# Autodesk Inventor assembly: Assembly1
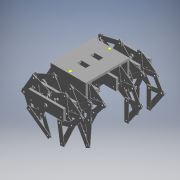
[picture p0: Inventor's stored thumbnail of the model, 180x180]
Saved by Autodesk Inventor 2018 (Build 220112000, 112)
## iProperties
Created: 2018-10-06
Part Number: Assembly1
Document SubType Name: Assembly
Designer: Jayden
Author: Jayden
## Documents named in this file (16)
- C:\Users\Jayden\Documents\Inventor\strandabeast\Assembly1.iam
- C:\Users\Jayden\Documents\Inventor\strandabeast\structural.ipt
- C:\Users\Jayden\Documents\Inventor\strandabeast\coupler.ipt
- C:\Users\Jayden\Documents\Inventor\strandabeast\crank bar.ipt
- C:\Users\Jayden\Documents\Inventor\strandabeast\Part B.ipt
- C:\Users\Jayden\Documents\Inventor\strandabeast\Part C.ipt
- C:\Users\Jayden\Documents\Inventor\strandabeast\Part D.ipt
- C:\Users\Jayden\Documents\Inventor\strandabeast\Part E.ipt
- C:\Users\Jayden\Documents\Inventor\strandabeast\Part F.ipt
- C:\Users\Jayden\Documents\Inventor\strandabeast\Part G.ipt
- C:\Users\Jayden\Documents\Inventor\strandabeast\Part H.ipt
- C:\Users\Jayden\Documents\Inventor\strandabeast\Part I.ipt
- C:\Users\Jayden\Documents\Inventor\strandabeast\Part J.ipt
- C:\Users\Jayden\Documents\Inventor\strandabeast\Part K.ipt
- C:\Users\Jayden\Documents\Inventor\strandabeast\structural small.ipt
- C:\Users\Jayden\Documents\Inventor\strandabeast\top.ipt
## Components (155 placed, 15 different names)
1. coupler:1 — Insert:3, Angle:3, Rotational:42
2. coupler:2 — Insert:1, Angle:1, Insert:2, Rotational:10, Rotational:11, Rotational:18, Rotational:19
3. coupler:3 — Rotational:39, Angle:42, Rotational:40, Angle:43, Rotational:41
4. crank bar:1 — Insert:1, Angle:1, Rotational:40, Angle:43
5. crank bar:2 — Insert:2, Insert:3, Angle:3
6. Part B:1 — Mate:12, Rotational:7, Angle:7, Angle:9
7. Part C:1 — Rotational:3, Rotational:6, Angle:12, Rotational:9, Mate:52
8. Part D:1 — Rotational:5, Rotational:6, Mate:11, Mate:12, Angle:7, Angle:8, Angle:9, Angle:10
9. Part E:1 — Mate:11, Rotational:8, Angle:10
10. Part F:1 — Rotational:4, Rotational:5, Angle:6, Angle:8
11. Part G:1 — Mate:8, Mate:9, Rotational:3, Rotational:4, Angle:4, Angle:5, Angle:6, Angle:11, Angle:12
12. Part H:1 — Mate:8, Angle:4, Angle:11, Mate:13, Angle:13
13. Part I:1 — Mate:9, Angle:5, Mate:13
14. Part J:1 — Rotational:7, Rotational:8, Rotational:10
15. Part K:1 — Rotational:9, Rotational:11
16. Part B:2 — Mate:25, Angle:18, Mate:26, Mate:54
17. Part C:2 — Rotational:12, Rotational:13, Angle:17, Rotational:17
18. Part D:2 — Mate:24, Rotational:13, Mate:25, Angle:18, Angle:19, Rotational:14
19. Part E:2 — Mate:24, Angle:19, Rotational:16
20. Part F:2 — Rotational:14, Rotational:15
21. Part G:2 — Mate:20, Mate:21, Angle:14, Angle:15, Angle:16, Rotational:12, Angle:17, Rotational:15
22. Part H:2 — Mate:21, Angle:14, Angle:16, Mate:22, Angle:20
23. Part I:2 — Mate:20, Angle:15, Mate:22
24. Part J:2 — Rotational:16, Mate:26, Rotational:18
25. Part K:2 — Rotational:17, Rotational:19
26. coupler:5 — Angle:40, Angle:41
27. coupler:6 — Rotational:61, Angle:61
28. crank bar:3 — Angle:41
29. crank bar:4 — Angle:40, Rotational:39, Angle:42
30. Part B:3
31. Part C:3 — Mate:53
32. Part D:3
33. Part E:3
34. Part F:3
35. Part G:3
36. Part H:3
37. Part I:3
38. Part J:3
39. Part K:3
40. Part B:4
41. Part C:4
42. Part D:4 — Mate:48
43. Part E:4
44. Part F:4
45. Part G:4
46. Part H:4
47. Part I:4
48. Part J:4
49. Part K:4
50. structural:3 — Mate:48, Mate:49, Mate:57, Mate:69, Mate:70, Mate:120, Mate:123, Mate:124
51. structural small:1 — Rotational:41, Mate:49, Mate:50, Mate:51, Mate:53, Mate:118
52. structural small:2 — Rotational:42, Mate:50, Mate:51, Mate:52, Mate:54, Mate:55, Mate:56
53. coupler:7
54. coupler:8 — Rotational:62
55. crank bar:5
56. crank bar:6 — Rotational:61, Angle:61
57. Part B:5
58. Part C:5
59. Part D:5 — Mate:70, Mate:72
60. Part E:5
61. Part F:5
62. Part G:5
63. Part H:5
64. Part I:5
65. Part J:5
66. Part K:5
67. Part B:6 — Mate:71
68. Part C:6 — Mate:69
69. Part D:6
70. Part E:6
71. Part F:6
72. Part G:6
73. Part H:6
74. Part I:6
75. Part J:6
76. Part K:6
77. structural small:3 — Rotational:62, Mate:71, Mate:72, Mate:119
78. coupler:9
79. coupler:10
80. coupler:11
81. crank bar:7
82. crank bar:8
83. Part B:7
84. Part C:7
85. Part D:7
86. Part E:7
87. Part F:7
88. Part G:7
89. Part H:7
90. Part I:7
91. Part J:7
92. Part K:7
93. Part B:8
94. Part C:8
95. Part D:8
96. Part E:8
97. Part F:8
98. Part G:8
99. Part H:8
100. Part I:8
101. Part J:8
102. Part K:8
103. coupler:12
104. coupler:13
105. crank bar:9
106. crank bar:10
107. Part B:9
108. Part C:9
109. Part D:9
110. Part E:9
111. Part F:9
112. Part G:9
113. Part H:9
114. Part I:9
115. Part J:9
116. Part K:9
117. Part B:10
118. Part C:10
119. Part D:10
120. Part E:10
121. Part F:10
122. Part G:10
123. Part H:10
124. Part I:10
125. Part J:10
126. Part K:10
127. structural:4 — Mate:121, Mate:122, Mate:125
128. structural small:4
129. structural small:5
130. coupler:14
131. coupler:15
132. crank bar:11
133. crank bar:12
134. Part B:11
135. Part C:11
136. Part D:11
137. Part E:11
138. Part F:11
139. Part G:11
140. Part H:11
141. Part I:11
142. Part J:11
143. Part K:11
144. Part B:12
145. Part C:12
146. Part D:12
147. Part E:12
148. Part F:12
149. Part G:12
150. Part H:12
151. Part I:12
152. Part J:12
153. Part K:12
154. structural small:6 — Mate:118, Mate:119
155. top:1 — Mate:120, Mate:121, Mate:122, Mate:123, Mate:124, Mate:125
## Relationships (349: RevoluteJoint 118, Angle 114, Mate 101, Insert 16)
- Insert:1 (-0.2794 mm): coupler:2 ↔ crank bar:1
- Angle:1 (180 deg): coupler:2 ↔ crank bar:1
- Insert:2 (-0.2794 mm): coupler:2 ↔ crank bar:2
- Insert:3: coupler:1 ↔ crank bar:2
- Angle:3 (0 deg): coupler:1 ↔ crank bar:2
- Mate:8: Part G:1 ↔ Part H:1
- Mate:9: Part G:1 ↔ Part I:1
- Rotational:3 [RevoluteJoint]: Part C:1 ↔ Part G:1
- Rotational:4 [RevoluteJoint]: Part F:1 ↔ Part G:1
- Rotational:5 [RevoluteJoint]: Part D:1 ↔ Part F:1
- Rotational:6 [RevoluteJoint]: Part C:1 ↔ Part D:1
- Mate:11: Part D:1 ↔ Part E:1
- Mate:12: Part B:1 ↔ Part D:1
- Rotational:7 [RevoluteJoint]: Part B:1 ↔ Part J:1
- Rotational:8 [RevoluteJoint]: Part E:1 ↔ Part J:1
- Angle:4 (0 deg): Part G:1 ↔ Part H:1
- Angle:5 (0 deg): Part G:1 ↔ Part I:1
- Angle:6 (0 deg): Part F:1 ↔ Part G:1
- Angle:7 (0 deg): Part B:1 ↔ Part D:1
- Angle:8 (0 deg): Part D:1 ↔ Part F:1
- Angle:9 (0 deg): Part B:1 ↔ Part D:1
- Angle:10 (0 deg): Part D:1 ↔ Part E:1
- Angle:11 (0 deg): Part G:1 ↔ Part H:1
- Angle:12 (0 deg): Part C:1 ↔ Part G:1
- Rotational:9 [RevoluteJoint]: Part C:1 ↔ Part K:1
- Mate:13: Part H:1 ↔ Part I:1
- Angle:13 (0 deg): Part H:1
- Rotational:10 [RevoluteJoint] (1.5875 mm): coupler:2 ↔ Part J:1
- Rotational:11 [RevoluteJoint] (-1.5875 mm): coupler:2 ↔ Part K:1
- Mate:20: Part G:2 ↔ Part I:2
- Mate:21: Part G:2 ↔ Part H:2
- Angle:14 (0 deg): Part G:2 ↔ Part H:2
- Angle:15 (0 deg): Part G:2 ↔ Part I:2
- Angle:16 (0 deg): Part G:2 ↔ Part H:2
- Mate:22: Part H:2 ↔ Part I:2
- Mate:24: Part D:2 ↔ Part E:2
- Rotational:12 [RevoluteJoint]: Part C:2 ↔ Part G:2
- Rotational:13 [RevoluteJoint]: Part C:2 ↔ Part D:2
- Angle:17 (0 deg): Part C:2 ↔ Part G:2
- Mate:25: Part B:2 ↔ Part D:2
- Angle:18 (0 deg): Part B:2 ↔ Part D:2
- Angle:19 (0 deg): Part D:2 ↔ Part E:2
- Rotational:14 [RevoluteJoint]: Part D:2 ↔ Part F:2
- Rotational:15 [RevoluteJoint]: Part F:2 ↔ Part G:2
- Rotational:16 [RevoluteJoint]: Part E:2 ↔ Part J:2
- Mate:26: Part B:2 ↔ Part J:2
- Rotational:17 [RevoluteJoint]: Part C:2 ↔ Part K:2
- Angle:20 (0 deg): Part H:2
- Rotational:18 [RevoluteJoint]: coupler:2 ↔ Part J:2
- Rotational:19 [RevoluteJoint] (3.175 mm): coupler:2 ↔ Part K:2
- [Insert] (-0.2794 mm): coupler:5 ↔ crank bar:3
- [Angle] (180 deg): coupler:5 ↔ crank bar:3
- [Insert] (-0.2794 mm): coupler:5 ↔ crank bar:4
- [Insert]: coupler:6 ↔ crank bar:3
- [Angle] (0 deg): coupler:6 ↔ crank bar:3
- [RevoluteJoint]: coupler:6 ↔ structural:3
- [Mate]: Part G:3 ↔ Part H:3
- [Mate]: Part G:3 ↔ Part I:3
- [RevoluteJoint]: Part C:3 ↔ Part G:3
- [RevoluteJoint]: Part F:3 ↔ Part G:3
- [RevoluteJoint]: Part D:3 ↔ Part F:3
- [RevoluteJoint]: Part C:3 ↔ Part D:3
- [Mate]: Part D:3 ↔ Part E:3
- [Mate]: Part B:3 ↔ Part D:3
- [RevoluteJoint]: Part B:3 ↔ Part J:3
- [RevoluteJoint]: Part E:3 ↔ Part J:3
- [Angle] (0 deg): Part G:3 ↔ Part H:3
- [Angle] (0 deg): Part G:3 ↔ Part I:3
- [Angle] (0 deg): Part F:3 ↔ Part G:3
- [Angle] (0 deg): Part B:3 ↔ Part D:3
- [Angle] (0 deg): Part D:3 ↔ Part F:3
- [Angle] (0 deg): Part B:3 ↔ Part D:3
- [Angle] (0 deg): Part D:3 ↔ Part E:3
- [Angle] (0 deg): Part G:3 ↔ Part H:3
- [Angle] (0 deg): Part C:3 ↔ Part G:3
- [RevoluteJoint]: Part C:3 ↔ Part K:3
- [Mate]: Part H:3 ↔ Part I:3
- [RevoluteJoint] (1.5875 mm): coupler:5 ↔ Part J:3
- [Mate]: Part C:3 ↔ structural:3
- [RevoluteJoint] (-1.5875 mm): coupler:5 ↔ Part K:3
- [Mate]: Part G:4 ↔ Part I:4
- [Mate]: Part G:4 ↔ Part H:4
- [Angle] (0 deg): Part G:4 ↔ Part H:4
- [Angle] (0 deg): Part G:4 ↔ Part I:4
- [Angle] (0 deg): Part G:4 ↔ Part H:4
- [Mate]: Part H:4 ↔ Part I:4
- [Mate]: Part D:4 ↔ Part E:4
- [RevoluteJoint]: Part C:4 ↔ Part G:4
- [RevoluteJoint]: Part C:4 ↔ Part D:4
- [Angle] (0 deg): Part C:4 ↔ Part G:4
- [Mate]: Part B:4 ↔ Part D:4
- [Angle] (0 deg): Part B:4 ↔ Part D:4
- [Angle] (0 deg): Part D:4 ↔ Part E:4
- [RevoluteJoint]: Part D:4 ↔ Part F:4
- [RevoluteJoint]: Part F:4 ↔ Part G:4
- [RevoluteJoint]: Part E:4 ↔ Part J:4
- [Mate]: Part B:4 ↔ Part J:4
- [RevoluteJoint]: Part C:4 ↔ Part K:4
- [RevoluteJoint]: coupler:5 ↔ Part J:4
- [RevoluteJoint] (3.175 mm): coupler:5 ↔ Part K:4
- Mate:48: Part D:4 ↔ structural:3
- Angle:40 (180 deg): coupler:5 ↔ crank bar:4
- Angle:41 (180 deg): coupler:5 ↔ crank bar:3
- Rotational:39 [RevoluteJoint]: coupler:3 ↔ crank bar:4
- Angle:42 (0 deg): coupler:3 ↔ crank bar:4
- Rotational:40 [RevoluteJoint]: coupler:3 ↔ crank bar:1
- Angle:43 (120 deg): coupler:3 ↔ crank bar:1
- Rotational:41 [RevoluteJoint]: coupler:3 ↔ structural small:1
- Rotational:42 [RevoluteJoint]: coupler:1 ↔ structural small:2
- Mate:49: structural:3 ↔ structural small:1
- Mate:50: structural small:1 ↔ structural small:2
- Mate:51: structural small:1 ↔ structural small:2
- Mate:52: Part C:1 ↔ structural small:2
- Mate:53: Part C:3 ↔ structural small:1
- Mate:54: Part B:2 ↔ structural small:2
- Mate:55: structural small:2
- Mate:56: structural small:2
- Mate:57: structural:3
- [Insert] (-0.2794 mm): coupler:7 ↔ crank bar:5
- [Angle] (180 deg): coupler:7 ↔ crank bar:5
- [Insert] (-0.2794 mm): coupler:7 ↔ crank bar:6
- [Mate]: Part G:5 ↔ Part H:5
- [Mate]: Part G:5 ↔ Part I:5
- [RevoluteJoint]: Part C:5 ↔ Part G:5
- [RevoluteJoint]: Part F:5 ↔ Part G:5
- [RevoluteJoint]: Part D:5 ↔ Part F:5
- [RevoluteJoint]: Part C:5 ↔ Part D:5
- [Mate]: Part D:5 ↔ Part E:5
- [Mate]: Part B:5 ↔ Part D:5
- [RevoluteJoint]: Part B:5 ↔ Part J:5
- [RevoluteJoint]: Part E:5 ↔ Part J:5
- [Angle] (0 deg): Part G:5 ↔ Part H:5
- [Angle] (0 deg): Part G:5 ↔ Part I:5
- [Angle] (0 deg): Part F:5 ↔ Part G:5
- [Angle] (0 deg): Part B:5 ↔ Part D:5
- [Angle] (0 deg): Part D:5 ↔ Part F:5
- [Angle] (0 deg): Part B:5 ↔ Part D:5
- [Angle] (0 deg): Part D:5 ↔ Part E:5
- [Angle] (0 deg): Part G:5 ↔ Part H:5
- [Angle] (0 deg): Part C:5 ↔ Part G:5
- [RevoluteJoint]: Part C:5 ↔ Part K:5
- [Mate]: Part H:5 ↔ Part I:5
- [RevoluteJoint] (1.5875 mm): coupler:7 ↔ Part J:5
- [RevoluteJoint] (-1.5875 mm): coupler:7 ↔ Part K:5
- [Mate]: Part G:6 ↔ Part I:6
- [Mate]: Part G:6 ↔ Part H:6
- [Angle] (0 deg): Part G:6 ↔ Part H:6
- [Angle] (0 deg): Part G:6 ↔ Part I:6
- [Angle] (0 deg): Part G:6 ↔ Part H:6
- [Mate]: Part H:6 ↔ Part I:6
- [Mate]: Part D:6 ↔ Part E:6
- [RevoluteJoint]: Part C:6 ↔ Part G:6
- [RevoluteJoint]: Part C:6 ↔ Part D:6
- [Angle] (0 deg): Part C:6 ↔ Part G:6
- [Mate]: Part B:6 ↔ Part D:6
- [Angle] (0 deg): Part B:6 ↔ Part D:6
- [Angle] (0 deg): Part D:6 ↔ Part E:6
- [RevoluteJoint]: Part D:6 ↔ Part F:6
- [RevoluteJoint]: Part F:6 ↔ Part G:6
- [RevoluteJoint]: Part E:6 ↔ Part J:6
- [Mate]: Part B:6 ↔ Part J:6
- [RevoluteJoint]: Part C:6 ↔ Part K:6
- [RevoluteJoint]: coupler:7 ↔ Part J:6
- [RevoluteJoint] (3.175 mm): coupler:7 ↔ Part K:6
- [RevoluteJoint]: coupler:8 ↔ crank bar:5
- [Angle] (120 deg): coupler:8 ↔ crank bar:5
- Rotational:61 [RevoluteJoint]: coupler:6 ↔ crank bar:6
- Mate:69: structural:3 ↔ Part C:6
- Mate:70: structural:3 ↔ Part D:5
- Rotational:62 [RevoluteJoint]: coupler:8 ↔ structural small:3
- Mate:71: Part B:6 ↔ structural small:3
- Mate:72: Part D:5 ↔ structural small:3
- Angle:61 (-120 deg): coupler:6 ↔ crank bar:6
- [Insert] (-0.2794 mm): coupler:10 ↔ crank bar:7
- [Angle] (180 deg): coupler:10 ↔ crank bar:7
- [Insert] (-0.2794 mm): coupler:10 ↔ crank bar:8
- [Insert]: coupler:9 ↔ crank bar:8
- [Angle] (0 deg): coupler:9 ↔ crank bar:8
- [Mate]: Part G:7 ↔ Part H:7
- [Mate]: Part G:7 ↔ Part I:7
- [RevoluteJoint]: Part C:7 ↔ Part G:7
- [RevoluteJoint]: Part F:7 ↔ Part G:7
- [RevoluteJoint]: Part D:7 ↔ Part F:7
- [RevoluteJoint]: Part C:7 ↔ Part D:7
- [Mate]: Part D:7 ↔ Part E:7
- [Mate]: Part B:7 ↔ Part D:7
- [RevoluteJoint]: Part B:7 ↔ Part J:7
- [RevoluteJoint]: Part E:7 ↔ Part J:7
- [Angle] (0 deg): Part G:7 ↔ Part H:7
- [Angle] (0 deg): Part G:7 ↔ Part I:7
- [Angle] (0 deg): Part F:7 ↔ Part G:7
- [Angle] (0 deg): Part B:7 ↔ Part D:7
- [Angle] (0 deg): Part D:7 ↔ Part F:7
- [Angle] (0 deg): Part B:7 ↔ Part D:7
- [Angle] (0 deg): Part D:7 ↔ Part E:7
- [Angle] (0 deg): Part G:7 ↔ Part H:7
- [Angle] (0 deg): Part C:7 ↔ Part G:7
- [RevoluteJoint]: Part C:7 ↔ Part K:7
- [Mate]: Part H:7 ↔ Part I:7
- [RevoluteJoint] (1.5875 mm): coupler:10 ↔ Part J:7
- [RevoluteJoint] (-1.5875 mm): coupler:10 ↔ Part K:7
- [Mate]: Part G:8 ↔ Part I:8
- [Mate]: Part G:8 ↔ Part H:8
- [Angle] (0 deg): Part G:8 ↔ Part H:8
- [Angle] (0 deg): Part G:8 ↔ Part I:8
- [Angle] (0 deg): Part G:8 ↔ Part H:8
- [Mate]: Part H:8 ↔ Part I:8
- [Mate]: Part D:8 ↔ Part E:8
- [RevoluteJoint]: Part C:8 ↔ Part G:8
- [RevoluteJoint]: Part C:8 ↔ Part D:8
- [Angle] (0 deg): Part C:8 ↔ Part G:8
- [Mate]: Part B:8 ↔ Part D:8
- [Angle] (0 deg): Part B:8 ↔ Part D:8
- [Angle] (0 deg): Part D:8 ↔ Part E:8
- [RevoluteJoint]: Part D:8 ↔ Part F:8
- [RevoluteJoint]: Part F:8 ↔ Part G:8
- [RevoluteJoint]: Part E:8 ↔ Part J:8
- [Mate]: Part B:8 ↔ Part J:8
- [RevoluteJoint]: Part C:8 ↔ Part K:8
- [RevoluteJoint]: coupler:10 ↔ Part J:8
- [RevoluteJoint] (3.175 mm): coupler:10 ↔ Part K:8
- [Insert] (-0.2794 mm): coupler:12 ↔ crank bar:9
- [Angle] (180 deg): coupler:12 ↔ crank bar:9
- [Insert] (-0.2794 mm): coupler:12 ↔ crank bar:10
- [Insert]: coupler:13 ↔ crank bar:9
- [Angle] (0 deg): coupler:13 ↔ crank bar:9
- [RevoluteJoint]: coupler:13 ↔ structural:4
- [Mate]: Part G:9 ↔ Part H:9
- [Mate]: Part G:9 ↔ Part I:9
- [RevoluteJoint]: Part C:9 ↔ Part G:9
- [RevoluteJoint]: Part F:9 ↔ Part G:9
- [RevoluteJoint]: Part D:9 ↔ Part F:9
- [RevoluteJoint]: Part C:9 ↔ Part D:9
- [Mate]: Part D:9 ↔ Part E:9
- [Mate]: Part B:9 ↔ Part D:9
- [RevoluteJoint]: Part B:9 ↔ Part J:9
- [RevoluteJoint]: Part E:9 ↔ Part J:9
- [Angle] (0 deg): Part G:9 ↔ Part H:9
- [Angle] (0 deg): Part G:9 ↔ Part I:9
- [Angle] (0 deg): Part F:9 ↔ Part G:9
- [Angle] (0 deg): Part B:9 ↔ Part D:9
- [Angle] (0 deg): Part D:9 ↔ Part F:9
- [Angle] (0 deg): Part B:9 ↔ Part D:9
- [Angle] (0 deg): Part D:9 ↔ Part E:9
- [Angle] (0 deg): Part G:9 ↔ Part H:9
- [Angle] (0 deg): Part C:9 ↔ Part G:9
- [RevoluteJoint]: Part C:9 ↔ Part K:9
- [Mate]: Part H:9 ↔ Part I:9
- [RevoluteJoint] (1.5875 mm): coupler:12 ↔ Part J:9
- [Mate]: Part C:9 ↔ structural:4
- [RevoluteJoint] (-1.5875 mm): coupler:12 ↔ Part K:9
- [Mate]: Part G:10 ↔ Part I:10
- [Mate]: Part G:10 ↔ Part H:10
- [Angle] (0 deg): Part G:10 ↔ Part H:10
- [Angle] (0 deg): Part G:10 ↔ Part I:10
- [Angle] (0 deg): Part G:10 ↔ Part H:10
- [Mate]: Part H:10 ↔ Part I:10
- [Mate]: Part D:10 ↔ Part E:10
- [RevoluteJoint]: Part C:10 ↔ Part G:10
- [RevoluteJoint]: Part C:10 ↔ Part D:10
- [Angle] (0 deg): Part C:10 ↔ Part G:10
- [Mate]: Part B:10 ↔ Part D:10
- [Angle] (0 deg): Part B:10 ↔ Part D:10
- [Angle] (0 deg): Part D:10 ↔ Part E:10
- [RevoluteJoint]: Part D:10 ↔ Part F:10
- [RevoluteJoint]: Part F:10 ↔ Part G:10
- [RevoluteJoint]: Part E:10 ↔ Part J:10
- [Mate]: Part B:10 ↔ Part J:10
- [RevoluteJoint]: Part C:10 ↔ Part K:10
- [RevoluteJoint]: coupler:12 ↔ Part J:10
- [RevoluteJoint] (3.175 mm): coupler:12 ↔ Part K:10
- [Mate]: Part D:10 ↔ structural:4
- [Angle] (180 deg): coupler:12 ↔ crank bar:10
- [Angle] (180 deg): coupler:12 ↔ crank bar:9
- [RevoluteJoint]: coupler:11 ↔ crank bar:10
- [Angle] (0 deg): coupler:11 ↔ crank bar:10
- [RevoluteJoint]: coupler:11 ↔ crank bar:7
- [Angle] (120 deg): coupler:11 ↔ crank bar:7
- [RevoluteJoint]: coupler:11 ↔ structural small:4
- [RevoluteJoint]: coupler:9 ↔ structural small:5
- [Mate]: structural:4 ↔ structural small:4
- [Mate]: structural small:4 ↔ structural small:5
- [Mate]: structural small:4 ↔ structural small:5
- [Mate]: Part C:7 ↔ structural small:5
- [Mate]: Part C:9 ↔ structural small:4
- [Mate]: Part B:8 ↔ structural small:5
- [Insert] (-0.2794 mm): coupler:14 ↔ crank bar:11
- [Angle] (180 deg): coupler:14 ↔ crank bar:11
- [Insert] (-0.2794 mm): coupler:14 ↔ crank bar:12
- [Mate]: Part G:11 ↔ Part H:11
- [Mate]: Part G:11 ↔ Part I:11
- [RevoluteJoint]: Part C:11 ↔ Part G:11
- [RevoluteJoint]: Part F:11 ↔ Part G:11
- [RevoluteJoint]: Part D:11 ↔ Part F:11
- [RevoluteJoint]: Part C:11 ↔ Part D:11
- [Mate]: Part D:11 ↔ Part E:11
- [Mate]: Part B:11 ↔ Part D:11
- [RevoluteJoint]: Part B:11 ↔ Part J:11
- [RevoluteJoint]: Part E:11 ↔ Part J:11
- [Angle] (0 deg): Part G:11 ↔ Part H:11
- [Angle] (0 deg): Part G:11 ↔ Part I:11
- [Angle] (0 deg): Part F:11 ↔ Part G:11
- [Angle] (0 deg): Part B:11 ↔ Part D:11
- [Angle] (0 deg): Part D:11 ↔ Part F:11
- [Angle] (0 deg): Part B:11 ↔ Part D:11
- [Angle] (0 deg): Part D:11 ↔ Part E:11
- [Angle] (0 deg): Part G:11 ↔ Part H:11
- [Angle] (0 deg): Part C:11 ↔ Part G:11
- [RevoluteJoint]: Part C:11 ↔ Part K:11
- [Mate]: Part H:11 ↔ Part I:11
- [RevoluteJoint] (1.5875 mm): coupler:14 ↔ Part J:11
- [RevoluteJoint] (-1.5875 mm): coupler:14 ↔ Part K:11
- [Mate]: Part G:12 ↔ Part I:12
- [Mate]: Part G:12 ↔ Part H:12
- [Angle] (0 deg): Part G:12 ↔ Part H:12
- [Angle] (0 deg): Part G:12 ↔ Part I:12
- [Angle] (0 deg): Part G:12 ↔ Part H:12
- [Mate]: Part H:12 ↔ Part I:12
- [Mate]: Part D:12 ↔ Part E:12
- [RevoluteJoint]: Part C:12 ↔ Part G:12
- [RevoluteJoint]: Part C:12 ↔ Part D:12
- [Angle] (0 deg): Part C:12 ↔ Part G:12
- [Mate]: Part B:12 ↔ Part D:12
- [Angle] (0 deg): Part B:12 ↔ Part D:12
- [Angle] (0 deg): Part D:12 ↔ Part E:12
- [RevoluteJoint]: Part D:12 ↔ Part F:12
- [RevoluteJoint]: Part F:12 ↔ Part G:12
- [RevoluteJoint]: Part E:12 ↔ Part J:12
- [Mate]: Part B:12 ↔ Part J:12
- [RevoluteJoint]: Part C:12 ↔ Part K:12
- [RevoluteJoint]: coupler:14 ↔ Part J:12
- [RevoluteJoint] (3.175 mm): coupler:14 ↔ Part K:12
- [RevoluteJoint]: coupler:15 ↔ crank bar:11
- [Angle] (120 deg): coupler:15 ↔ crank bar:11
- [RevoluteJoint]: coupler:13 ↔ crank bar:12
- [Mate]: structural:4 ↔ Part C:12
- [Mate]: structural:4 ↔ Part D:11
- [RevoluteJoint]: coupler:15 ↔ structural small:6
- [Mate]: Part B:12 ↔ structural small:6
- [Mate]: Part D:11 ↔ structural small:6
- [Angle] (-120 deg): coupler:13 ↔ crank bar:12
- Mate:118: structural small:1 ↔ structural small:6
- Mate:119: structural small:3 ↔ structural small:6
- Mate:120: structural:3 ↔ top:1
- Mate:121: structural:4 ↔ top:1
- Mate:122: structural:4 ↔ top:1
- Mate:123: structural:3 ↔ top:1
- Mate:124: structural:3 ↔ top:1
- Mate:125: structural:4 ↔ top:1
## Named parameters: d128_d99 = 0 mm, d129_d100 = -124.855953 deg, d130_d101 = 0 mm, d131_d102 = -121.340978 deg, d132_d103 = 0 deg, d133_d104 = 0 mm, d134_d105 = 0 deg, d135_d106 = 0 deg, d136_d113 = 0 mm, d137_d114 = 127.362564 deg, d138_d115 = 0 mm, d139_d116 = -49.122461 deg, d140_d117 = 0 mm, d141_d118 = 111.287823 deg, d142_d119 = 0 mm, d143_d120 = 0 mm, d144_d121 = 53.752768 deg, d145_d123 = 0 mm, d146_d124 = -171.93596 deg, d151_d91 = 0 mm, d152_d92 = 0 mm, d153_d93 = 0 deg, d154_d94 = 0 deg, d155_d95 = 0 deg, d156_d96 = 0 mm, d157_d98 = 0 mm, d158_d33 = 90.296984 deg, d159_d34 = 0 mm, d160_d35 = -89.375001 deg, d161_d36 = 0 mm, d162_d37 = 94.335322 deg, d163_d38 = 0 mm, d164_d39 = 0 mm, d165_d40 = 0 mm, d166_d41 = -133.774107 deg, d167_d42 = 0 mm, d168_d43 = -87.957363 deg, d169_d57 = 1.5875 mm, d170_d58 = -53.00241 deg, d171_d59 = 0 mm, d172_d60 = -1.5875 mm, d173_d61 = 35.472433 deg, d174_d44 = 0 deg, d175_d45 = 0 deg, d176_d46 = 0 deg, d177_d47 = 0 deg, d178_d48 = 0 deg, d179_d49 = 0 deg, d180_d50 = 0 deg, d181_d51 = 0 deg, d182_d52 = 0 deg, d183_d53 = 0 mm, d184_d54 = -145.818065 deg, d185_d55 = 0 mm, d188_d27 = 0 mm, d189_d28 = 0 mm, d190_d30 = 0 mm, d191_d31 = 94.663337 deg, d192_d32 = 0 mm, d194_d126 = 3.175 mm, d195_d127 = -83.550522 deg, d196_d14 = 0 deg, d198_d16 = 0 mm, d199_d17 = 153.57524 deg, d202_d0 = -0.2794 mm, d203_d1 = 180 deg, d204_d2 = -0.2794 mm, d206_d4 = 0 mm, d269_d253 = 0 mm, d270_d254 = -30 deg, d271_d255 = 120 deg, d272_d0 = -0.2794 mm, d273_d1 = 180 deg, d274_d2 = -0.2794 mm, d275_d113 = 0 mm, d276_d114 = 140.971398 deg, d277_d115 = 0 mm, d278_d116 = -33.195148 deg, d279_d117 = 0 mm, d280_d118 = 119.311328 deg, d281_d119 = 0 mm, d282_d120 = 0 mm, d283_d121 = 61.347796 deg, d284_d123 = 0 mm, d285_d124 = 99.003061 deg, d286_d126 = 3.175 mm, d287_d127 = -176.141747 deg, d288_d91 = 0 mm, d289_d92 = 0 mm, d290_d93 = 0 deg, d291_d94 = 0 deg, d292_d95 = 0 deg, d293_d96 = 0 mm, d294_d98 = 0 mm, d295_d99 = 0 mm, d296_d100 = -139.262717 deg, d297_d101 = 0 mm, d298_d102 = -133.429264 deg, d299_d103 = 0 deg, d300_d104 = 0 mm, d301_d105 = 0 deg, d302_d106 = 0 deg, d303_d57 = 1.5875 mm, d304_d58 = 146.705681 deg, d305_d60 = -1.5875 mm, d306_d61 = -125.094014 deg, d307_d34 = 0 mm, d308_d35 = -78.978121 deg, d309_d36 = 0 mm, d310_d37 = 83.967171 deg, d311_d38 = 0 mm, d312_d39 = 0 mm, d313_d40 = 0 mm, d314_d41 = -128.896709 deg, d315_d42 = 0 mm, d316_d43 = -83.079965 deg, d317_d44 = 0 deg, d318_d45 = 0 deg, d319_d46 = 0 deg, d320_d47 = 0 deg, d321_d48 = 0 deg, d322_d49 = 0 deg, d323_d50 = 0 deg, d324_d51 = 0 deg, d325_d52 = 0 deg, d326_d53 = 0 mm, d327_d54 = -140.601849 deg, d328_d55 = 0 mm, d329_d27 = 0 mm, d330_d28 = 0 mm, d331_d30 = 0 mm, d332_d31 = 83.328454 deg, d333_d32 = 0 mm, d334_d33 = 101.660596 deg, d356_d333_d32 = 0 mm, d357_d334_d33 = 68.554601 deg, d358_d269_d253 = 0 mm, d359_d270_d254 = -30 deg, d360_d271_d255 = 120 deg, d361_d272_d0 = -0.2794 mm, d362_d273_d1 = 180 deg, d363_d274_d2 = -0.2794 mm, d364_d275_d113 = 0 mm, d365_d276_d114 = 176.366301 deg, d366_d277_d115 = 0 mm, d367_d278_d116 = 110.22292 deg, d368_d279_d117 = 0 mm, d369_d280_d118 = -118.898194 deg, d370_d281_d119 = 0 mm, d371_d282_d120 = 0 mm, d372_d283_d121 = 60.962481 deg, d373_d284_d123 = 0 mm, d374_d285_d124 = -97.516884 deg, d375_d286_d126 = 3.175 mm, d376_d287_d127 = -105.089393 deg, d377_d288_d91 = 0 mm, d378_d289_d92 = 0 mm, d379_d290_d93 = 0 deg, d380_d291_d94 = 0 deg, d381_d292_d95 = 0 deg, d382_d293_d96 = 0 mm, d383_d294_d98 = 0 mm, d384_d295_d99 = 0 mm, d385_d296_d100 = 179.566551 deg, d386_d297_d101 = 0 mm, d387_d298_d102 = -66.57683 deg, d388_d299_d103 = 0 deg, d389_d300_d104 = 0 mm, d390_d301_d105 = 0 deg, d391_d302_d106 = 0 deg, d392_d303_d57 = 1.5875 mm, d393_d304_d58 = -84.082529 deg, d394_d305_d60 = -1.5875 mm, d395_d306_d61 = 7.703324 deg, d396_d307_d34 = 0 mm, d397_d308_d35 = -109.129533 deg, d398_d309_d36 = 0 mm, d399_d310_d37 = 114.570683 deg, d400_d311_d38 = 0 mm, d401_d312_d39 = 0 mm, d402_d313_d40 = 0 mm, d403_d314_d41 = -141.603916 deg, d404_d315_d42 = 0 mm, d405_d316_d43 = -95.787172 deg, d406_d317_d44 = 0 deg, d407_d318_d45 = 0 deg, d408_d319_d46 = 0 deg, d409_d320_d47 = 0 deg, d410_d321_d48 = 0 deg, d411_d322_d49 = 0 deg, d412_d323_d50 = 0 deg, d413_d324_d51 = 0 deg, d414_d325_d52 = 0 deg, d415_d326_d53 = 0 mm, d416_d327_d54 = -154.912605 deg, d417_d328_d55 = 0 mm, d418_d329_d27 = 0 mm, d419_d330_d28 = 0 mm, d420_d331_d30 = 0 mm, d421_d332_d31 = 116.886549 deg, d422_d258 = 0 mm, d423_d259 = -142.425382 deg, d424_d260 = 0 mm, d425_d261 = 0 mm, d426_d262 = 0 mm, d427_d263 = 0 mm, d428_d253 = 0 mm, d429_d254 = -30 deg, d430_d255 = 120 deg, d431_d256 = 0 mm, d432_d257 = -22.425382 deg, d433_d249 = 0 mm, d434_d250 = 90 deg, d435_d251 = 0 deg, d436_d355 = -120 deg, d437_d353 = 0 mm, d438_d354 = 0 mm, d439_d347 = 0 mm, d440_d348 = -150 deg, d441_d349 = 0 mm, d442_d350 = 0 mm, d443_d351 = 0 mm, d444_d352 = 67.574618 deg, d445_d0 = -0.2794 mm, d446_d1 = 180 deg, d447_d2 = -0.2794 mm, d448_d264 = 0 mm, d449_d265 = 0 mm, d450_d244 = 180 deg, d451_d245 = 180 deg, d452_d239 = 0 mm, d453_d128_d99 = 0 mm, d454_d129_d100 = -53.533513 deg, d455_d130_d101 = 0 mm, d456_d131_d102 = -56.85897 deg, d457_d132_d103 = 0 deg, d458_d133_d104 = 0 mm, d459_d134_d105 = 0 deg, d460_d135_d106 = 0 deg, d461_d136_d113 = 0 mm, d462_d137_d114 = 62.777236 deg, d463_d138_d115 = 0 mm, d464_d139_d116 = -120.548221 deg, d465_d140_d117 = 0 mm, d466_d141_d118 = 81.54096 deg, d467_d142_d119 = 0 mm, d468_d143_d120 = 0 mm, d469_d144_d121 = 21.622571 deg, d470_d145_d123 = 0 mm, d471_d146_d124 = -74.403609 deg, d472_d151_d91 = 0 mm, d473_d152_d92 = 0 mm, d474_d153_d93 = 0 deg, d475_d154_d94 = 0 deg, d476_d155_d95 = 0 deg, d477_d156_d96 = 0 mm, d478_d157_d98 = 0 mm, d479_d158_d33 = 152.851035 deg, d480_d159_d34 = 0 mm, d481_d160_d35 = -34.158478 deg, d482_d161_d36 = 0 mm, d483_d162_d37 = 42.599784 deg, d484_d163_d38 = 0 mm, d485_d164_d39 = 0 mm, d486_d165_d40 = 0 mm, d487_d166_d41 = -103.719206 deg, d488_d167_d42 = 0 mm, d489_d168_d43 = -57.902462 deg, d490_d169_d57 = 1.5875 mm, d491_d170_d58 = 20.594731 deg, d492_d171_d59 = 0 mm, d493_d172_d60 = -1.5875 mm, d494_d173_d61 = 117.138126 deg, d495_d174_d44 = 0 deg, d496_d175_d45 = 0 deg, d497_d176_d46 = 0 deg, d498_d177_d47 = 0 deg, d499_d178_d48 = 0 deg, d500_d179_d49 = 0 deg, d501_d180_d50 = 0 deg, d502_d181_d51 = 0 deg, d503_d182_d52 = 0 deg, d504_d183_d53 = 0 mm, d505_d184_d54 = -116.068875 deg, d506_d185_d55 = 0 mm, d507_d188_d27 = 0 mm, d508_d189_d28 = 0 mm, d509_d190_d30 = 0 mm, d510_d191_d31 = 35.590271 deg, d511_d192_d32 = 0 mm, d512_d194_d126 = 3.175 mm, d513_d195_d127 = 11.376882 deg, d514_d196_d14 = 0 deg, d515_d198_d16 = 0 mm, d516_d199_d17 = -112.425382 deg, d517_d202_d0 = -0.2794 mm, d518_d203_d1 = 180 deg, d519_d204_d2 = -0.2794 mm, d520_d206_d4 = 0 mm, d521_d113 = 0 mm, d522_d114 = 140.263429 deg, d523_d115 = 0 mm, d524_d116 = -34.053736 deg, d525_d117 = 0 mm, d526_d118 = 118.898194 deg, d527_d119 = 0 mm, d528_d120 = 0 mm, d529_d121 = 60.962481 deg, d530_d123 = 0 mm, d531_d124 = 169.854711 deg, d532_d126 = 3.175 mm, d533_d127 = -105.089393 deg, d534_d91 = 0 mm, d535_d92 = 0 mm, d536_d93 = 0 deg, d537_d94 = 0 deg, d538_d95 = 0 deg, d539_d96 = 0 mm, d540_d98 = 0 mm, d541_d99 = 0 mm, d542_d100 = -138.514354 deg, d543_d101 = 0 mm, d544_d102 = -132.831519 deg, d545_d103 = 0 deg, d546_d104 = 0 mm, d547_d105 = 0 deg, d548_d106 = 0 deg, d549_d57 = 1.5875 mm, d550_d58 = -84.082529 deg, d551_d60 = -1.5875 mm, d552_d61 = 7.703324 deg, d553_d34 = 0 mm, d554_d35 = -109.129533 deg, d555_d36 = 0 mm, d556_d37 = 114.570683 deg, d557_d38 = 0 mm, d558_d39 = 0 mm, d559_d40 = 0 mm, d560_d41 = -141.603916 deg, d561_d42 = 0 mm, d562_d43 = -95.787172 deg, d563_d44 = 0 deg, d564_d45 = 0 deg, d565_d46 = 0 deg, d566_d47 = 0 deg, d567_d48 = 0 deg, d568_d49 = 0 deg, d569_d50 = 0 deg, d570_d51 = 0 deg, d571_d52 = 0 deg, d572_d53 = 0 mm, d573_d54 = -154.912605 deg, d574_d55 = 0 mm, d575_d3 = 0 mm, d576_d15 = 0 deg, d577_d27 = 0 mm, d578_d28 = 0 mm, d579_d30 = 0 mm, d580_d31 = 116.886549 deg, d581_d32 = 0 mm, d582_d33 = 68.554601 deg
